# Autodesk Inventor assembly: Assembly
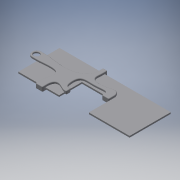
[picture p0: Inventor's stored thumbnail of the model, 180x180]
Saved by Autodesk Inventor 2018 (Build 220112000, 112)
## iProperties
Created: 2018-05-12
Part Number: Assembly
Document SubType Name: Assembly
Designer: Mandus
Author: Mandus
## Documents named in this file (3)
- C:\Users\Mandus\Dropbox\Skola\Projekt\Kretsn_Brillz_V2\3D\Ovve_Holder\Assembly.iam
- C:\Users\Mandus\Dropbox\Skola\Projekt\Kretsn_Brillz_V2\3D\Ovve_Holder\PCB.ipt
- C:\Users\Mandus\Dropbox\Skola\Projekt\Kretsn_Brillz_V2\3D\Ovve_Holder\Holder.ipt
## Components (2 placed, 2 different names)
1. PCB:1 — Flush:1
2. Holder:1 — Flush:1
## Relationships (1: Flush 1)
- Flush:1: PCB:1 ↔ Holder:1
